# Autodesk Inventor assembly: module_command
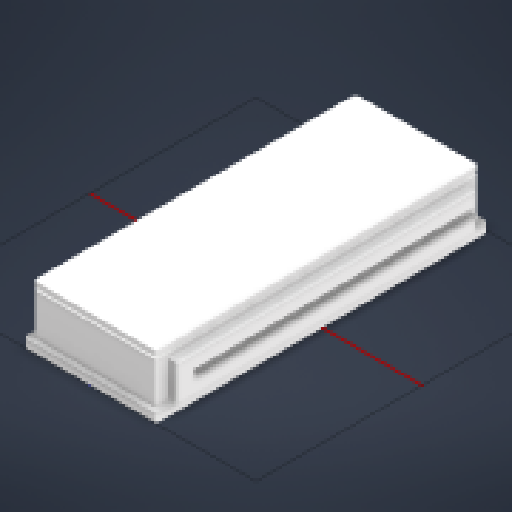
[picture p0: Inventor's stored thumbnail of the model, 512x512]
Saved by Autodesk Inventor 2025.2 (Build 292293000, 293)
## iProperties
Created: 2025-11-12
Part Number: module_command
Document SubType Name: Assembly
Designer: sam
Author: sam
## Documents named in this file (4)
- G:\projects\primary\regulated-irrigation-system\model\asm\module-command\module_command.iam
- G:\projects\primary\regulated-irrigation-system\model\asm\module-command\module_command.ipt
- G:\projects\primary\regulated-irrigation-system\model\asm\module-command\module-lid_command.ipt
- G:\projects\primary\regulated-irrigation-system\model\asm\module-command\electronics-command_perfboard.iam
## Components (3 placed, 3 different names)
1. module_command:1 — Mate:1, Mate:2, Mate:3, Mate:4, Mate:5
2. module-lid_command:1 — Mate:1, Mate:2
3. electronics-command_perfboard:1 [sub-assembly] — Mate:3, Mate:4, Mate:5
## Relationships (5: Mate 5)
- Mate:1: module_command:1 ↔ module-lid_command:1
- Mate:2: module_command:1 ↔ module-lid_command:1
- Mate:3: module_command:1 ↔ electronics-command_perfboard:1
- Mate:4: module_command:1 ↔ electronics-command_perfboard:1
- Mate:5: module_command:1 ↔ electronics-command_perfboard:1
